# Autodesk Inventor assembly: Enclosure
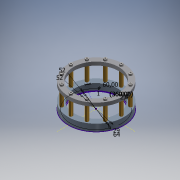
[picture p0: Inventor's stored thumbnail of the model, 180x180]
Saved by Autodesk Inventor 2018.3 (Build 223284000, 284)
## iProperties
Created: 2018-08-03
Part Number: Enclosure
Material: Generisch
Document SubType Name: Assembly
Designer: JochenAlt
Author: JochenAlt
## Documents named in this file (5)
- D:\Projects\FlowerPot\CAD\CycloidalGear2\Enclosure.iam
- D:\Projects\FlowerPot\CAD\CycloidalGear2\Enclosure.ipt
- D:\Projects\FlowerPot\CAD\CycloidalGear2\Roll.iam
- C:\Users\JochenAlt\Documents\Inventor\Content Center Files\R2018\de-DE\DIN 912\DIN 912 - M2 x 0,4 x 16 x 15.ipt
- C:\Users\JochenAlt\Documents\Inventor\Content Center Files\R2018\de-DE\DIN 912\DIN 912 - M2 x 0,4 x 12 x 11.ipt
## Components (37 placed, 4 different names)
1. Enclosure:1 — Passend:25, Passend:27, Passend:28, Passend:29, Passend:30, Passend:31, Passend:32, Passend:33, Passend:34, Passend:35, Passend:36, Passend:37, Einfügen:1, Einfügen:2, Einfügen:3, Einfügen:4, Einfügen:5, Einfügen:6, Einfügen:7, Einfügen:8, Einfügen:9, Einfügen:10, Einfügen:11, Einfügen:12, Einfügen:13, Einfügen:14, Einfügen:15, Einfügen:16, Einfügen:17, Einfügen:18, Einfügen:19, Einfügen:20, Einfügen:21, Einfügen:22, Einfügen:23, Einfügen:24, Passend:49, Passend:50, Passend:51, Passend:52, Passend:53, Passend:54, Passend:55, Passend:56, Passend:57, Passend:58, Passend:59, Passend:60
2. Roll:1 [sub-assembly] — Passend:36, Passend:49
3. Roll:2 [sub-assembly] — Passend:35, Passend:50
4. Roll:3 [sub-assembly] — Passend:37, Passend:51
5. Roll:4 [sub-assembly] — Passend:34, Passend:52
6. Roll:5 [sub-assembly] — Passend:33, Passend:53
7. Roll:6 [sub-assembly] — Passend:32, Passend:54
8. Roll:7 [sub-assembly] — Passend:27, Passend:55
9. Roll:8 [sub-assembly] — Passend:28, Passend:59
10. Roll:9 [sub-assembly] — Passend:29, Passend:58
11. Roll:10 [sub-assembly] — Passend:31, Passend:56
12. Roll:11 [sub-assembly] — Passend:25, Passend:60
13. Roll:12 [sub-assembly] — Passend:30, Passend:57
14. DIN 912 - ersetzt durch DIN EN ISO 4762 M2 x 16:1 — Einfügen:1
15. DIN 912 - ersetzt durch DIN EN ISO 4762 M2 x 16:2 — Einfügen:2
16. DIN 912 - ersetzt durch DIN EN ISO 4762 M2 x 16:3 — Einfügen:3
17. DIN 912 - ersetzt durch DIN EN ISO 4762 M2 x 16:4 — Einfügen:4
18. DIN 912 - ersetzt durch DIN EN ISO 4762 M2 x 16:5 — Einfügen:5
19. DIN 912 - ersetzt durch DIN EN ISO 4762 M2 x 16:6 — Einfügen:6
20. DIN 912 - ersetzt durch DIN EN ISO 4762 M2 x 16:7 — Einfügen:7
21. DIN 912 - ersetzt durch DIN EN ISO 4762 M2 x 16:8 — Einfügen:8
22. DIN 912 - ersetzt durch DIN EN ISO 4762 M2 x 16:9 — Einfügen:9
23. DIN 912 - ersetzt durch DIN EN ISO 4762 M2 x 16:10 — Einfügen:10
24. DIN 912 - ersetzt durch DIN EN ISO 4762 M2 x 16:11 — Einfügen:11
25. DIN 912 - ersetzt durch DIN EN ISO 4762 M2 x 16:12 — Einfügen:12
26. DIN 912 - ersetzt durch DIN EN ISO 4762 M2 x 12:1 — Einfügen:13
27. DIN 912 - ersetzt durch DIN EN ISO 4762 M2 x 12:2 — Einfügen:14
28. DIN 912 - ersetzt durch DIN EN ISO 4762 M2 x 12:3 — Einfügen:15
29. DIN 912 - ersetzt durch DIN EN ISO 4762 M2 x 12:4 — Einfügen:16
30. DIN 912 - ersetzt durch DIN EN ISO 4762 M2 x 12:5 — Einfügen:17
31. DIN 912 - ersetzt durch DIN EN ISO 4762 M2 x 12:6 — Einfügen:18
32. DIN 912 - ersetzt durch DIN EN ISO 4762 M2 x 12:7 — Einfügen:19
33. DIN 912 - ersetzt durch DIN EN ISO 4762 M2 x 12:8 — Einfügen:20
34. DIN 912 - ersetzt durch DIN EN ISO 4762 M2 x 12:9 — Einfügen:21
35. DIN 912 - ersetzt durch DIN EN ISO 4762 M2 x 12:10 — Einfügen:22
36. DIN 912 - ersetzt durch DIN EN ISO 4762 M2 x 12:11 — Einfügen:23
37. DIN 912 - ersetzt durch DIN EN ISO 4762 M2 x 12:12 — Einfügen:24
## Relationships (48: Mate 24, Insert 24)
- Passend:25 [Mate]: Enclosure:1 ↔ Roll:11
- Passend:27 [Mate]: Enclosure:1 ↔ Roll:7
- Passend:28 [Mate]: Enclosure:1 ↔ Roll:8
- Passend:29 [Mate]: Enclosure:1 ↔ Roll:9
- Passend:30 [Mate]: Enclosure:1 ↔ Roll:12
- Passend:31 [Mate]: Enclosure:1 ↔ Roll:10
- Passend:32 [Mate]: Enclosure:1 ↔ Roll:6
- Passend:33 [Mate]: Enclosure:1 ↔ Roll:5
- Passend:34 [Mate]: Enclosure:1 ↔ Roll:4
- Passend:35 [Mate]: Enclosure:1 ↔ Roll:2
- Passend:36 [Mate]: Enclosure:1 ↔ Roll:1
- Passend:37 [Mate]: Enclosure:1 ↔ Roll:3
- Einfügen:1 [Insert]: Enclosure:1 ↔ DIN 912 - ersetzt durch DIN EN ISO 4762 M2 x 16:1
- Einfügen:2 [Insert]: Enclosure:1 ↔ DIN 912 - ersetzt durch DIN EN ISO 4762 M2 x 16:2
- Einfügen:3 [Insert]: Enclosure:1 ↔ DIN 912 - ersetzt durch DIN EN ISO 4762 M2 x 16:3
- Einfügen:4 [Insert]: Enclosure:1 ↔ DIN 912 - ersetzt durch DIN EN ISO 4762 M2 x 16:4
- Einfügen:5 [Insert]: Enclosure:1 ↔ DIN 912 - ersetzt durch DIN EN ISO 4762 M2 x 16:5
- Einfügen:6 [Insert]: Enclosure:1 ↔ DIN 912 - ersetzt durch DIN EN ISO 4762 M2 x 16:6
- Einfügen:7 [Insert]: Enclosure:1 ↔ DIN 912 - ersetzt durch DIN EN ISO 4762 M2 x 16:7
- Einfügen:8 [Insert]: Enclosure:1 ↔ DIN 912 - ersetzt durch DIN EN ISO 4762 M2 x 16:8
- Einfügen:9 [Insert]: Enclosure:1 ↔ DIN 912 - ersetzt durch DIN EN ISO 4762 M2 x 16:9
- Einfügen:10 [Insert]: Enclosure:1 ↔ DIN 912 - ersetzt durch DIN EN ISO 4762 M2 x 16:10
- Einfügen:11 [Insert]: Enclosure:1 ↔ DIN 912 - ersetzt durch DIN EN ISO 4762 M2 x 16:11
- Einfügen:12 [Insert]: Enclosure:1 ↔ DIN 912 - ersetzt durch DIN EN ISO 4762 M2 x 16:12
- Einfügen:13 [Insert]: Enclosure:1 ↔ DIN 912 - ersetzt durch DIN EN ISO 4762 M2 x 12:1
- Einfügen:14 [Insert]: Enclosure:1 ↔ DIN 912 - ersetzt durch DIN EN ISO 4762 M2 x 12:2
- Einfügen:15 [Insert]: Enclosure:1 ↔ DIN 912 - ersetzt durch DIN EN ISO 4762 M2 x 12:3
- Einfügen:16 [Insert]: Enclosure:1 ↔ DIN 912 - ersetzt durch DIN EN ISO 4762 M2 x 12:4
- Einfügen:17 [Insert]: Enclosure:1 ↔ DIN 912 - ersetzt durch DIN EN ISO 4762 M2 x 12:5
- Einfügen:18 [Insert]: Enclosure:1 ↔ DIN 912 - ersetzt durch DIN EN ISO 4762 M2 x 12:6
- Einfügen:19 [Insert]: Enclosure:1 ↔ DIN 912 - ersetzt durch DIN EN ISO 4762 M2 x 12:7
- Einfügen:20 [Insert]: Enclosure:1 ↔ DIN 912 - ersetzt durch DIN EN ISO 4762 M2 x 12:8
- Einfügen:21 [Insert]: Enclosure:1 ↔ DIN 912 - ersetzt durch DIN EN ISO 4762 M2 x 12:9
- Einfügen:22 [Insert]: Enclosure:1 ↔ DIN 912 - ersetzt durch DIN EN ISO 4762 M2 x 12:10
- Einfügen:23 [Insert]: Enclosure:1 ↔ DIN 912 - ersetzt durch DIN EN ISO 4762 M2 x 12:11
- Einfügen:24 [Insert]: Enclosure:1 ↔ DIN 912 - ersetzt durch DIN EN ISO 4762 M2 x 12:12
- Passend:49 [Mate]: Enclosure:1 ↔ Roll:1
- Passend:50 [Mate]: Enclosure:1 ↔ Roll:2
- Passend:51 [Mate]: Enclosure:1 ↔ Roll:3
- Passend:52 [Mate]: Enclosure:1 ↔ Roll:4
- Passend:53 [Mate]: Enclosure:1 ↔ Roll:5
- Passend:54 [Mate]: Enclosure:1 ↔ Roll:6
- Passend:55 [Mate]: Enclosure:1 ↔ Roll:7
- Passend:56 [Mate]: Enclosure:1 ↔ Roll:10
- Passend:57 [Mate]: Enclosure:1 ↔ Roll:12
- Passend:58 [Mate]: Enclosure:1 ↔ Roll:9
- Passend:59 [Mate]: Enclosure:1 ↔ Roll:8
- Passend:60 [Mate]: Enclosure:1 ↔ Roll:11
